# Autodesk Inventor assembly: V2 Gantry
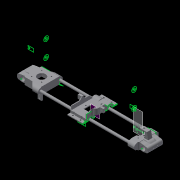
[picture p0: Inventor's stored thumbnail of the model, 180x180]
Saved by Autodesk Inventor 2014 (Build 180170000, 170)
## iProperties
Created: 2015-07-07
Part Number: V2 Gantry
Document SubType Name: Assembly
Designer: Scott
Author: Scott
## Documents named in this file (5)
- C:\Users\Scott\Google Drive\Engineering Ideas and Designs\3D printer\PISCES\PISCES_(IPTandSTL)\Parts (IPTandSTL)\IPTs\V2 Gantry.iam
- C:\Users\Scott\Google Drive\Engineering Ideas and Designs\3D printer\PISCES\PISCES_(IPTandSTL)\Parts (IPTandSTL)\IPTs\Xcarriage Left V2.ipt
- C:\Users\Scott\Documents\footbar.ipt
- C:\Users\Scott\Google Drive\Engineering Ideas and Designs\3D printer\PISCES\PISCES_(IPTandSTL)\Parts (IPTandSTL)\IPTs\Xcarriage Left V2_MIR.ipt
- C:\Users\Scott\Google Drive\Engineering Ideas and Designs\3D printer\PISCES\PISCES_(IPTandSTL)\Parts (IPTandSTL)\IPTs\Extruder Holder V2.ipt
## Components (4 placed, 4 different names)
1. Xcarriage Left V2:1 — Flush:1
2. footbar:1 — Flush:1, Mate:1
3. Xcarriage Left V2_MIR:1 — Mate:1
4. Extruder Holder V2:1 — Flush:2, Flush:3
## Relationships (4: Flush 3, Mate 1)
- Flush:1: Xcarriage Left V2:1 ↔ footbar:1
- Mate:1: footbar:1 ↔ Xcarriage Left V2_MIR:1
- Flush:2: Extruder Holder V2:1
- Flush:3: Extruder Holder V2:1
